# Autodesk Inventor assembly: A_Wing
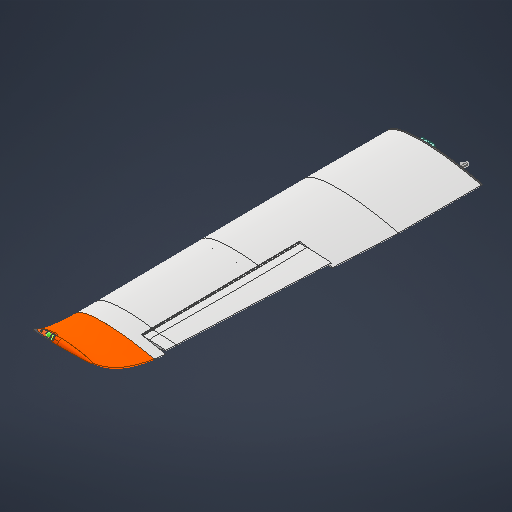
[picture p0: Inventor's stored thumbnail of the model, 512x512]
Saved by Autodesk Inventor 2026 (Build 300175000, 175)
## iProperties
Created: 2025-09-10
Part Number: A_Wing
Document SubType Name: Assembly
Designer: FAL
Author: FAL
## iProperties of the stored document MemberDocs/xU5ojcpinBkx0hnfkLeo1mnbp5e
Created: 2025-09-10
Part Number: A_Wing
Document SubType Name: Assembly
Designer: FAL
Author: FAL
## Documents named in this file (17)
- C:\Users\FAL\Projekte\Git\AIRBERT\CAD\Wing\A_Wing.iam
- C:\Users\FAL\Projekte\Git\AIRBERT\CAD\Wing\P_Wing_aileron_lever.ipt
- C:\Users\FAL\Projekte\Git\AIRBERT\CAD\Wing\P_Wing_inner.ipt
- C:\Users\FAL\Projekte\Git\AIRBERT\CAD\Wing\P_Wing_mid.ipt
- C:\Users\FAL\Projekte\Git\AIRBERT\CAD\Wing\P_Wing_mid_servocap.ipt
- C:\Users\FAL\Projekte\Git\AIRBERT\CAD\Wing\P_Wing_mid_servolink.ipt
- C:\Users\FAL\Projekte\Git\AIRBERT\CAD\Wing\P_Wing_Mountingplate.ipt
- C:\Users\FAL\Projekte\Git\AIRBERT\CAD\Wing\P_Wing_winglet.ipt
- C:\Users\FAL\Projekte\Git\AIRBERT\CAD\Wing\P_Wing_winglet_LEDcap.ipt
- C:\Users\FAL\Projekte\Git\AIRBERT\CAD\Wing\P_Wing_aileron.ipt
- C:\Users\FAL\Projekte\Git\AIRBERT\CAD\Electronic\P_JX9_F_ref.ipt
- C:\Users\FAL\Projekte\Git\AIRBERT\CAD\Electronic\P_LED_5.ipt
- C:\Users\FAL\Projekte\Git\AIRBERT\CAD\Electronic\P_Servo_SIMPROP.ipt
- C:\Users\FAL\Projekte\Git\AIRBERT\CAD\Electronic\P_Servo_SIMPROP_lever.ipt
- C:\Users\FAL\Projekte\Git\AIRBERT\CAD\Wing\P_Wing.ipt
- C:\Users\FAL\Projekte\Git\AIRBERT\CAD\Wing\P_Wing_Mountingplate_pin.ipt
- C:\Users\FAL\Projekte\Git\AIRBERT\CAD\Wing\P_Wing_inner_add.ipt
## Components (16 placed, 16 different names)
1. P_Wing_mid_servolink:1 — Passend:18, Tangential:1, Passend:19
2. P_Wing_inner:1 — Fluchtend:1, Fluchtend:2, Fluchtend:3, Passend:9, Passend:10, Passend:11, Passend:23, Passend:24
3. P_Wing_mid:1 — Fluchtend:4, Fluchtend:5, Fluchtend:6, Passend:16, Passend:26
4. P_Wing_mid_servocap:1 — Fluchtend:7, Fluchtend:8, Fluchtend:9
5. P_Wing_Mountingplate:1 — Fluchtend:10, Fluchtend:11, Fluchtend:12, Passend:20, Passend:21, Passend:25, Fluchtend:24, Passend:27
6. P_Wing_winglet:1 — Fluchtend:13, Fluchtend:14, Fluchtend:15
7. P_Wing_winglet_LEDcap:1 — Fluchtend:16, Fluchtend:17, Fluchtend:18, Passend:8, Passend:12
8. P_Wing_aileron:1 — Passend:13, Passend:14, Passend:15, Passend:16, Passend:26
9. P_Wing_aileron_lever:1 — Passend:13, Passend:14, Passend:15, Tangential:1
10. P_Wing_Mountingplate_pin:1 — Passend:23, Passend:24, Passend:25
11. P_Wing_inner_add:1 — Fluchtend:25, Fluchtend:26, Fluchtend:27, Passend:27
12. P_JX9_F_ref:1 — Passend:20, Passend:21, Fluchtend:24
13. P_LED_5:1 — Passend:8, Passend:12
14. P_Servo_SIMPROP:1 — Passend:5, Passend:6, Passend:9, Passend:10, Passend:11
15. P_Servo_SIMPROP_lever:1 — Passend:5, Passend:6, Passend:18, Passend:19
16. P_Wing:1 — Fluchtend:21, Fluchtend:22, Fluchtend:23
## Relationships (46: Flush 25, Mate 20, Tangent 1)
- Fluchtend:1 [Flush]: P_Wing_inner:1
- Fluchtend:2 [Flush]: P_Wing_inner:1
- Fluchtend:3 [Flush]: P_Wing_inner:1
- Fluchtend:4 [Flush]: P_Wing_mid:1
- Fluchtend:5 [Flush]: P_Wing_mid:1
- Fluchtend:6 [Flush]: P_Wing_mid:1
- Fluchtend:7 [Flush]: P_Wing_mid_servocap:1
- Fluchtend:8 [Flush]: P_Wing_mid_servocap:1
- Fluchtend:9 [Flush]: P_Wing_mid_servocap:1
- Fluchtend:10 [Flush]: P_Wing_Mountingplate:1
- Fluchtend:11 [Flush]: P_Wing_Mountingplate:1
- Fluchtend:12 [Flush]: P_Wing_Mountingplate:1
- Fluchtend:13 [Flush]: P_Wing_winglet:1
- Fluchtend:14 [Flush]: P_Wing_winglet:1
- Fluchtend:15 [Flush]: P_Wing_winglet:1
- Fluchtend:16 [Flush]: P_Wing_winglet_LEDcap:1
- Fluchtend:17 [Flush]: P_Wing_winglet_LEDcap:1
- Fluchtend:18 [Flush]: P_Wing_winglet_LEDcap:1
- Passend:5 [Mate]: P_Servo_SIMPROP:1 ↔ P_Servo_SIMPROP_lever:1
- Passend:6 [Mate]: P_Servo_SIMPROP:1 ↔ P_Servo_SIMPROP_lever:1
- Passend:8 [Mate]: P_Wing_winglet_LEDcap:1 ↔ P_LED_5:1
- Passend:9 [Mate]: P_Wing_inner:1 ↔ P_Servo_SIMPROP:1
- Passend:10 [Mate]: P_Wing_inner:1 ↔ P_Servo_SIMPROP:1
- Passend:11 [Mate]: P_Wing_inner:1 ↔ P_Servo_SIMPROP:1
- Passend:12 [Mate]: P_Wing_winglet_LEDcap:1 ↔ P_LED_5:1
- Fluchtend:21 [Flush]: P_Wing:1
- Fluchtend:22 [Flush]: P_Wing:1
- Fluchtend:23 [Flush]: P_Wing:1
- Passend:13 [Mate]: P_Wing_aileron:1 ↔ P_Wing_aileron_lever:1
- Passend:14 [Mate] (0.25 mm): P_Wing_aileron:1 ↔ P_Wing_aileron_lever:1
- Passend:15 [Mate] (0.2525 mm): P_Wing_aileron:1 ↔ P_Wing_aileron_lever:1
- Passend:16 [Mate]: P_Wing_mid:1 ↔ P_Wing_aileron:1
- Passend:18 [Mate]: P_Wing_mid_servolink:1 ↔ P_Servo_SIMPROP_lever:1
- Tangential:1: P_Wing_mid_servolink:1 ↔ P_Wing_aileron_lever:1
- Passend:19 [Mate]: P_Wing_mid_servolink:1 ↔ P_Servo_SIMPROP_lever:1
- Passend:20 [Mate] (0.5 mm): P_Wing_Mountingplate:1 ↔ P_JX9_F_ref:1
- Passend:21 [Mate] (1.5 mm): P_Wing_Mountingplate:1 ↔ P_JX9_F_ref:1
- Passend:23 [Mate] (0.1 mm): P_Wing_inner:1 ↔ P_Wing_Mountingplate_pin:1
- Passend:24 [Mate] (0.1 mm): P_Wing_inner:1 ↔ P_Wing_Mountingplate_pin:1
- Passend:25 [Mate] (7.5 mm): P_Wing_Mountingplate:1 ↔ P_Wing_Mountingplate_pin:1
- Passend:26 [Mate]: P_Wing_mid:1 ↔ P_Wing_aileron:1
- Fluchtend:24 [Flush]: P_Wing_Mountingplate:1 ↔ P_JX9_F_ref:1
- Fluchtend:25 [Flush]: P_Wing_inner_add:1
- Fluchtend:26 [Flush]: P_Wing_inner_add:1
- Fluchtend:27 [Flush]: P_Wing_inner_add:1
- Passend:27 [Mate]: P_Wing_Mountingplate:1 ↔ P_Wing_inner_add:1
